# Autodesk Inventor assembly: GFRP_T2_20
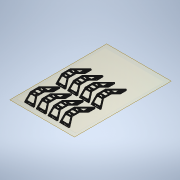
[picture p0: Inventor's stored thumbnail of the model, 180x180]
Saved by Autodesk Inventor 2020 (Build 240168000, 168)
## iProperties
Created: 2021-08-27
Part Number: GFRP_T2_20
Document SubType Name: Assembly
Designer: Masato
Author: Masato
## Documents named in this file (3)
- C:\Inventor\SUSTAINA-OP\Cam\GFRP_T2_20.iam
- C:\Inventor\SUSTAINA-OP\Cam\DisposableBoard.ipt
- C:\Inventor\SUSTAINA-OP\UpperBody\Head\Head_side_frame.ipt
## Components (9 placed, 2 different names)
1. DisposableBoard:1 — メイト:2, メイト:1, フラッシュ:1, フラッシュ:2, メイト:5, フラッシュ:3, フラッシュ:4
2. Head_side_frame:2 — メイト:5, フラッシュ:3, フラッシュ:4
3. Head_side_frame:3
4. Head_side_frame:4
5. Head_side_frame:5
6. Head_side_frame:6
7. Head_side_frame:7
8. Head_side_frame:8
9. Head_side_frame:9
## Component patterns: (2 elements), (4 elements, first: Head_side_frame:2), コンポーネント パターン 4:2 (4 elements)
## Relationships (7: Flush 4, Mate 3)
- メイト:2 [Mate]: DisposableBoard:1
- メイト:1 [Mate]: DisposableBoard:1
- フラッシュ:1 [Flush]: DisposableBoard:1
- フラッシュ:2 [Flush]: DisposableBoard:1
- メイト:5 [Mate]: DisposableBoard:1 ↔ Head_side_frame:2
- フラッシュ:3 [Flush] (2 mm): DisposableBoard:1 ↔ Head_side_frame:2
- フラッシュ:4 [Flush] (2 mm): DisposableBoard:1 ↔ Head_side_frame:2
